# Autodesk Inventor assembly: rv_ledbrick_8ch
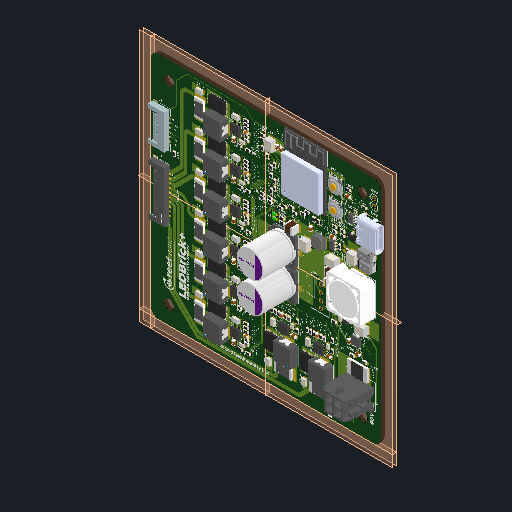
[picture p0: Inventor's stored thumbnail of the model, 512x512]
Saved by Autodesk Inventor 2026.1 (Build 301233020, 233B)
## iProperties
Created: 2025-09-11
Part Number: rv_ledbrick_8ch
Document SubType Name: Assembly
Designer: atrus
Author: atrus
## Documents named in this file (49)
- C:\Users\atrus\Dropbox\elec\Mechanical\LEDBrick\PCB\rv_ledbrick_8ch.iam
- C:\Users\atrus\Dropbox\elec\Mechanical\LEDBrick\PCB\rv_ledbrick_8ch_BOARD.ipt
- C:\Users\atrus\Dropbox\elec\Mechanical\LEDBrick\PCB\ConvertedComponents\LED_WS2812B2020_CMP-004-00042-1.ipt
- C:\Users\atrus\Dropbox\elec\Mechanical\LEDBrick\PCB\ConvertedComponents\RESC1608-IPC-ML_CMP-009-00193-3.ipt
- C:\Users\atrus\Dropbox\elec\Mechanical\LEDBrick\PCB\ConvertedComponents\SOT23-3_CMP-094-0000-1.ipt
- C:\Users\atrus\Dropbox\elec\Mechanical\LEDBrick\PCB\ConvertedComponents\RESC1608-IPC-LL_CMP-009-00205-1.ipt
- C:\Users\atrus\Dropbox\elec\Mechanical\LEDBrick\PCB\ConvertedComponents\RESC1608-IPC-NL_CMP-009-00180-2.ipt
- C:\Users\atrus\Dropbox\elec\Mechanical\LEDBrick\PCB\ConvertedComponents\RESC1608-IPC-ML_CMP-009-00191-4.ipt
- C:\Users\atrus\Dropbox\elec\Mechanical\LEDBrick\PCB\ConvertedComponents\RESC1608-IPC-NL_CMP-009-00191-4.ipt
- C:\Users\atrus\Dropbox\elec\Mechanical\LEDBrick\PCB\ConvertedComponents\FP-DGS0010A-IPC_C_CMP-015-00018-1.ipt
- C:\Users\atrus\Dropbox\elec\Mechanical\LEDBrick\PCB\ConvertedComponents\FP-RC0603-0_55-MFG_CMP-009-00246-1.ipt
- C:\Users\atrus\Dropbox\elec\Mechanical\LEDBrick\PCB\ConvertedComponents\RESC7146X09N_CMP-009-00241-2.ipt
- C:\Users\atrus\Dropbox\elec\Mechanical\LEDBrick\PCB\ConvertedComponents\FP-43045-0428-MFG_CMP-002-00096-1.ipt
- C:\Users\atrus\Dropbox\elec\Mechanical\LEDBrick\PCB\ConvertedComponents\FP-CL10-IPC_B_CMP-001-00084-7.ipt
- C:\Users\atrus\Dropbox\elec\Mechanical\LEDBrick\PCB\ConvertedComponents\LED-0603_CMP-130-0000-1.ipt
- C:\Users\atrus\Dropbox\elec\Mechanical\LEDBrick\PCB\ConvertedComponents\FP-504050-1091-MFG_CMP-002-00088-1.ipt
- C:\Users\atrus\Dropbox\elec\Mechanical\LEDBrick\PCB\ConvertedComponents\MOLEX_5040500691_CMP-253-000000-2.ipt
- C:\Users\atrus\Dropbox\elec\Mechanical\LEDBrick\PCB\ConvertedComponents\FP-OS-CON-SMT-F12-MFG_CMP-001-00120-1.ipt
- C:\Users\atrus\Dropbox\elec\Mechanical\LEDBrick\PCB\ConvertedComponents\SOT95P280X145-6N_CMP-019-00077-1.ipt
- C:\Users\atrus\Dropbox\elec\Mechanical\LEDBrick\PCB\ConvertedComponents\FP-DDC0006A-IPC_C_CMP-019-00081-1.ipt
- C:\Users\atrus\Dropbox\elec\Mechanical\LEDBrick\PCB\ConvertedComponents\XCVR_ESP32-S3-MINI-1-N8_CMP-247-000000-1.ipt
- C:\Users\atrus\Dropbox\elec\Mechanical\LEDBrick\PCB\ConvertedComponents\FP-PTS526SK15SMTR2LFS-MFG_CMP-011-00015-1.ipt
- C:\Users\atrus\Dropbox\elec\Mechanical\LEDBrick\PCB\ConvertedComponents\RESC1608X55X30NL20T20_CMP-009-00235-1.ipt
- C:\Users\atrus\Dropbox\elec\Mechanical\LEDBrick\PCB\ConvertedComponents\RESC1608-IPC-LL_CMP-009-00203-1.ipt
- C:\Users\atrus\Dropbox\elec\Mechanical\LEDBrick\PCB\ConvertedComponents\RESC1608-IPC-LL_CMP-009-00207-3.ipt
- C:\Users\atrus\Dropbox\elec\Mechanical\LEDBrick\PCB\ConvertedComponents\FP-AC0402-IPC_A_CMP-009-00234-1.ipt
- C:\Users\atrus\Dropbox\elec\Mechanical\LEDBrick\PCB\ConvertedComponents\SRR1260-680M-Footprint-1_CMP-006-00034-1.ipt
- C:\Users\atrus\Dropbox\elec\Mechanical\LEDBrick\PCB\ConvertedComponents\FP-SRN4018-MFG_CMP-006-00036-2.ipt
- C:\Users\atrus\Dropbox\elec\Mechanical\LEDBrick\PCB\ConvertedComponents\AMPHENOL_10155435-00011LF_CMP-243-000000-3.ipt
- C:\Users\atrus\Dropbox\elec\Mechanical\LEDBrick\PCB\ConvertedComponents\SMA_CMP-080-0002-2.ipt
- C:\Users\atrus\Dropbox\elec\Mechanical\LEDBrick\PCB\ConvertedComponents\FP-SOT23-6L-MFG_CMP-004-00040-1.ipt
- C:\Users\atrus\Dropbox\elec\Mechanical\LEDBrick\PCB\ConvertedComponents\CAPC3225X20N_CMP-001-00083-3.ipt
- C:\Users\atrus\Dropbox\elec\Mechanical\LEDBrick\PCB\ConvertedComponents\FP-1210-L_3_2_0_3-W_2_5_0-MFG_CMP-001-00125-1.ipt
- C:\Users\atrus\Dropbox\elec\Mechanical\LEDBrick\PCB\ConvertedComponents\CAPC1210(3225)230_M_CMP-001-00128-1.ipt
- C:\Users\atrus\Dropbox\elec\Mechanical\LEDBrick\PCB\ConvertedComponents\FP-GRM32E-0_2-0_3-MFG_CMP-001-00119-1.ipt
- C:\Users\atrus\Dropbox\elec\Mechanical\LEDBrick\PCB\ConvertedComponents\CAPC2013X94X50ML20T25_CMP-001-00130-1.ipt
- C:\Users\atrus\Dropbox\elec\Mechanical\LEDBrick\PCB\ConvertedComponents\FP-CL10-IPC_B_CMP-001-00085-7.ipt
- C:\Users\atrus\Dropbox\elec\Mechanical\LEDBrick\PCB\ConvertedComponents\RESC1608-IPC-NL_CMP-009-00208-2.ipt
- C:\Users\atrus\Dropbox\elec\Mechanical\LEDBrick\PCB\ConvertedComponents\SON50P300X100_HS-13N_CMP-019-00085-2.ipt
- C:\Users\atrus\Dropbox\elec\Mechanical\LEDBrick\PCB\ConvertedComponents\RESC1608-IPC-NL_CMP-009-00203-1.ipt
- C:\Users\atrus\Dropbox\elec\Mechanical\LEDBrick\PCB\ConvertedComponents\RESC1608X55X30ML15T15_CMP-009-00245-1.ipt
- C:\Users\atrus\Dropbox\elec\Mechanical\LEDBrick\PCB\ConvertedComponents\FP-CRCW0603-e3-IPC_B_CMP-009-00244-2.ipt
- C:\Users\atrus\Dropbox\elec\Mechanical\LEDBrick\PCB\ConvertedComponents\RESC1608-IPC-NL_CMP-009-00187-4.ipt
- C:\Users\atrus\Dropbox\elec\Mechanical\LEDBrick\PCB\ConvertedComponents\RESC1608-IPC-NL_CMP-009-00193-3.ipt
- C:\Users\atrus\Dropbox\elec\Mechanical\LEDBrick\PCB\ConvertedComponents\FP-CRA2512-MFG_CMP-009-00243-1.ipt
- C:\Users\atrus\Dropbox\elec\Mechanical\LEDBrick\PCB\ConvertedComponents\FP-IHLP-2525CZ-FP_2_413x3-MFG_CMP-006-00037-1.ipt
- C:\Users\atrus\Dropbox\elec\Mechanical\LEDBrick\PCB\ConvertedComponents\DFN355P580X82-3N_CMP-004-00041-2.ipt
- C:\Users\atrus\Dropbox\elec\Mechanical\LEDBrick\PCB\ConvertedComponents\FP-0603-L_1_6_0_15-W_0_81-IPC_B_CMP-001-00131-2.ipt
- C:\Users\atrus\Dropbox\elec\Mechanical\LEDBrick\PCB\ConvertedComponents\CAPC2013X94X50NL20T25_CMP-001-00130-1.ipt
## Components (210 placed, 210 different names)
1. rv_ledbrick_8ch_BOARD:1 — Symmetry:1, Symmetry:2
2. LED_WS2812B2020_CMP-004-00042-1:1{D200}
3. RESC1608-IPC-ML_CMP-009-00193-3:1{R230}
4. RESC1608-IPC-ML_CMP-009-00193-3:2{R205}
5. RESC1608-IPC-ML_CMP-009-00193-3:3{R206}
6. SOT23-3_CMP-094-0000-1:1{Q201}
7. SOT23-3_CMP-094-0000-1:2{Q200}
8. RESC1608-IPC-LL_CMP-009-00205-1:1{R10}
9. RESC1608-IPC-NL_CMP-009-00180-2:1{R229}
10. RESC1608-IPC-NL_CMP-009-00180-2:2{R228}
11. RESC1608-IPC-NL_CMP-009-00180-2:3{R224}
12. RESC1608-IPC-NL_CMP-009-00180-2:4{R9_H}
13. RESC1608-IPC-NL_CMP-009-00180-2:5{R9_G}
14. RESC1608-IPC-NL_CMP-009-00180-2:6{R9_F}
15. RESC1608-IPC-NL_CMP-009-00180-2:7{R9_E}
16. RESC1608-IPC-NL_CMP-009-00180-2:8{R9_D}
17. RESC1608-IPC-NL_CMP-009-00180-2:9{R9_C}
18. RESC1608-IPC-NL_CMP-009-00180-2:10{R9_B}
19. RESC1608-IPC-NL_CMP-009-00180-2:11{R9_A}
20. RESC1608-IPC-NL_CMP-009-00180-2:12{R8_H}
21. RESC1608-IPC-NL_CMP-009-00180-2:13{R8_G}
22. RESC1608-IPC-NL_CMP-009-00180-2:14{R8_F}
23. RESC1608-IPC-NL_CMP-009-00180-2:15{R8_E}
24. RESC1608-IPC-NL_CMP-009-00180-2:16{R8_D}
25. RESC1608-IPC-NL_CMP-009-00180-2:17{R8_C}
26. RESC1608-IPC-NL_CMP-009-00180-2:18{R8_B}
27. RESC1608-IPC-NL_CMP-009-00180-2:19{R8_A}
28. RESC1608-IPC-ML_CMP-009-00191-4:1{R227}
29. RESC1608-IPC-ML_CMP-009-00191-4:2{R226}
30. RESC1608-IPC-ML_CMP-009-00191-4:3{R223}
31. RESC1608-IPC-ML_CMP-009-00191-4:4{R222}
32. RESC1608-IPC-ML_CMP-009-00191-4:5{R221}
33. RESC1608-IPC-ML_CMP-009-00191-4:6{R204}
34. RESC1608-IPC-ML_CMP-009-00191-4:7{R202}
35. RESC1608-IPC-ML_CMP-009-00191-4:8{R201}
36. RESC1608-IPC-NL_CMP-009-00191-4:1{R225}
37. RESC1608-IPC-NL_CMP-009-00191-4:2{R220}
38. RESC1608-IPC-NL_CMP-009-00191-4:3{R219}
39. RESC1608-IPC-NL_CMP-009-00191-4:4{R218}
40. RESC1608-IPC-NL_CMP-009-00191-4:5{R217}
41. RESC1608-IPC-NL_CMP-009-00191-4:6{R216}
42. RESC1608-IPC-NL_CMP-009-00191-4:7{R215}
43. RESC1608-IPC-NL_CMP-009-00191-4:8{R214}
44. RESC1608-IPC-NL_CMP-009-00191-4:9{R213}
45. RESC1608-IPC-NL_CMP-009-00191-4:10{R212}
46. RESC1608-IPC-NL_CMP-009-00191-4:11{R211}
47. RESC1608-IPC-NL_CMP-009-00191-4:12{R210}
48. RESC1608-IPC-NL_CMP-009-00191-4:13{R209}
49. RESC1608-IPC-NL_CMP-009-00191-4:14{R208}
50. RESC1608-IPC-NL_CMP-009-00191-4:15{R207}
51. RESC1608-IPC-NL_CMP-009-00191-4:16{R203}
52. RESC1608-IPC-NL_CMP-009-00191-4:17{R200}
53. FP-DGS0010A-IPC_C_CMP-015-00018-1:1{U500}
54. FP-RC0603-0_55-MFG_CMP-009-00246-1:1{R502}
55. FP-RC0603-0_55-MFG_CMP-009-00246-1:2{R500}
56. RESC7146X09N_CMP-009-00241-2:1{R501}
57. FP-43045-0428-MFG_CMP-002-00096-1:1{J500}
58. FP-CL10-IPC_B_CMP-001-00084-7:1{C501}
59. FP-CL10-IPC_B_CMP-001-00084-7:2{C500}
60. FP-CL10-IPC_B_CMP-001-00084-7:3{C404}
61. FP-CL10-IPC_B_CMP-001-00084-7:4{C401}
62. FP-CL10-IPC_B_CMP-001-00084-7:5{C201}
63. FP-CL10-IPC_B_CMP-001-00084-7:6{C200}
64. LED-0603_CMP-130-0000-1:1{LED201}
65. LED-0603_CMP-130-0000-1:2{LED200}
66. FP-504050-1091-MFG_CMP-002-00088-1:1{J4}
67. FP-504050-1091-MFG_CMP-002-00088-1:2{J1}
68. MOLEX_5040500691_CMP-253-000000-2:1{J3}
69. FP-OS-CON-SMT-F12-MFG_CMP-001-00120-1:1{C6}
70. FP-OS-CON-SMT-F12-MFG_CMP-001-00120-1:2{C5}
71. SOT95P280X145-6N_CMP-019-00077-1:1{U400}
72. FP-DDC0006A-IPC_C_CMP-019-00081-1:1{U401}
73. XCVR_ESP32-S3-MINI-1-N8_CMP-247-000000-1:1{U200}
74. FP-PTS526SK15SMTR2LFS-MFG_CMP-011-00015-1:1{RST200}
75. FP-PTS526SK15SMTR2LFS-MFG_CMP-011-00015-1:2{BOOT200}
76. RESC1608X55X30NL20T20_CMP-009-00235-1:1{R402}
77. RESC1608-IPC-LL_CMP-009-00203-1:1{R400}
78. RESC1608-IPC-LL_CMP-009-00203-1:2{R401}
79. RESC1608-IPC-LL_CMP-009-00207-3:1{R403}
80. FP-AC0402-IPC_A_CMP-009-00234-1:1{R301}
81. FP-AC0402-IPC_A_CMP-009-00234-1:2{R300}
82. SRR1260-680M-Footprint-1_CMP-006-00034-1:1{L400}
83. FP-SRN4018-MFG_CMP-006-00036-2:1{L401}
84. AMPHENOL_10155435-00011LF_CMP-243-000000-3:1{J300}
85. SMA_CMP-080-0002-2:1{D401}
86. SMA_CMP-080-0002-2:2{D400}
87. FP-SOT23-6L-MFG_CMP-004-00040-1:1{D300}
88. CAPC3225X20N_CMP-001-00083-3:1{C410}
89. CAPC3225X20N_CMP-001-00083-3:2{C402}
90. CAPC3225X20N_CMP-001-00083-3:3{C405}
91. CAPC3225X20N_CMP-001-00083-3:4{C202}
92. FP-1210-L_3_2_0_3-W_2_5_0-MFG_CMP-001-00125-1:1{C409}
93. FP-1210-L_3_2_0_3-W_2_5_0-MFG_CMP-001-00125-1:2{C403}
94. CAPC1210(3225)230_M_CMP-001-00128-1:1{C406}
95. FP-GRM32E-0_2-0_3-MFG_CMP-001-00119-1:1{C407}
96. CAPC2013X94X50ML20T25_CMP-001-00130-1:1{C400}
97. FP-CL10-IPC_B_CMP-001-00085-7:1{C206}
98. FP-CL10-IPC_B_CMP-001-00085-7:2{C203}
99. FP-CL10-IPC_B_CMP-001-00085-7:3{C2_H}
100. FP-CL10-IPC_B_CMP-001-00085-7:4{C2_G}
101. FP-CL10-IPC_B_CMP-001-00085-7:5{C2_F}
102. FP-CL10-IPC_B_CMP-001-00085-7:6{C2_E}
103. FP-CL10-IPC_B_CMP-001-00085-7:7{C2_D}
104. FP-CL10-IPC_B_CMP-001-00085-7:8{C2_C}
105. FP-CL10-IPC_B_CMP-001-00085-7:9{C2_B}
106. FP-CL10-IPC_B_CMP-001-00085-7:10{C2_A}
107. RESC1608-IPC-NL_CMP-009-00208-2:1{R4_F}
108. RESC1608-IPC-NL_CMP-009-00208-2:2{R4_H}
109. RESC1608-IPC-NL_CMP-009-00208-2:3{R4_G}
110. RESC1608-IPC-NL_CMP-009-00208-2:4{R4_E}
111. RESC1608-IPC-NL_CMP-009-00208-2:5{R4_D}
112. RESC1608-IPC-NL_CMP-009-00208-2:6{R4_C}
113. RESC1608-IPC-NL_CMP-009-00208-2:7{R4_B}
114. RESC1608-IPC-NL_CMP-009-00208-2:8{R4_A}
115. SON50P300X100_HS-13N_CMP-019-00085-2:1{U1_H}
116. SON50P300X100_HS-13N_CMP-019-00085-2:2{U1_G}
117. SON50P300X100_HS-13N_CMP-019-00085-2:3{U1_F}
118. SON50P300X100_HS-13N_CMP-019-00085-2:4{U1_E}
119. SON50P300X100_HS-13N_CMP-019-00085-2:5{U1_D}
120. SON50P300X100_HS-13N_CMP-019-00085-2:6{U1_C}
121. SON50P300X100_HS-13N_CMP-019-00085-2:7{U1_B}
122. SON50P300X100_HS-13N_CMP-019-00085-2:8{U1_A}
123. RESC1608-IPC-NL_CMP-009-00203-1:1{R7_H}
124. RESC1608-IPC-NL_CMP-009-00203-1:2{R7_G}
125. RESC1608-IPC-NL_CMP-009-00203-1:3{R7_F}
126. RESC1608-IPC-NL_CMP-009-00203-1:4{R7_E}
127. RESC1608-IPC-NL_CMP-009-00203-1:5{R7_D}
128. RESC1608-IPC-NL_CMP-009-00203-1:6{R7_C}
129. RESC1608-IPC-NL_CMP-009-00203-1:7{R7_B}
130. RESC1608-IPC-NL_CMP-009-00203-1:8{R7_A}
131. RESC1608X55X30ML15T15_CMP-009-00245-1:1{R6_H}
132. RESC1608X55X30ML15T15_CMP-009-00245-1:2{R6_G}
133. RESC1608X55X30ML15T15_CMP-009-00245-1:3{R6_F}
134. RESC1608X55X30ML15T15_CMP-009-00245-1:4{R6_E}
135. RESC1608X55X30ML15T15_CMP-009-00245-1:5{R6_D}
136. RESC1608X55X30ML15T15_CMP-009-00245-1:6{R6_C}
137. RESC1608X55X30ML15T15_CMP-009-00245-1:7{R6_B}
138. RESC1608X55X30ML15T15_CMP-009-00245-1:8{R6_A}
139. FP-CRCW0603-e3-IPC_B_CMP-009-00244-2:1{R5_H}
140. FP-CRCW0603-e3-IPC_B_CMP-009-00244-2:2{R5_G}
141. FP-CRCW0603-e3-IPC_B_CMP-009-00244-2:3{R5_F}
142. FP-CRCW0603-e3-IPC_B_CMP-009-00244-2:4{R5_E}
143. FP-CRCW0603-e3-IPC_B_CMP-009-00244-2:5{R5_D}
144. FP-CRCW0603-e3-IPC_B_CMP-009-00244-2:6{R5_C}
145. FP-CRCW0603-e3-IPC_B_CMP-009-00244-2:7{R5_B}
146. FP-CRCW0603-e3-IPC_B_CMP-009-00244-2:8{R5_A}
147. RESC1608-IPC-NL_CMP-009-00187-4:1{R3_H}
148. RESC1608-IPC-NL_CMP-009-00187-4:2{R3_G}
149. RESC1608-IPC-NL_CMP-009-00187-4:3{R3_F}
150. RESC1608-IPC-NL_CMP-009-00187-4:4{R3_E}
151. RESC1608-IPC-NL_CMP-009-00187-4:5{R3_D}
152. RESC1608-IPC-NL_CMP-009-00187-4:6{R3_C}
153. RESC1608-IPC-NL_CMP-009-00187-4:7{R3_B}
154. RESC1608-IPC-NL_CMP-009-00187-4:8{R3_A}
155. RESC1608-IPC-NL_CMP-009-00193-3:1{R2_H}
156. RESC1608-IPC-NL_CMP-009-00193-3:2{R2_G}
157. RESC1608-IPC-NL_CMP-009-00193-3:3{R2_F}
158. RESC1608-IPC-NL_CMP-009-00193-3:4{R2_E}
159. RESC1608-IPC-NL_CMP-009-00193-3:5{R2_D}
160. RESC1608-IPC-NL_CMP-009-00193-3:6{R2_C}
161. RESC1608-IPC-NL_CMP-009-00193-3:7{R2_B}
162. RESC1608-IPC-NL_CMP-009-00193-3:8{R2_A}
163. FP-CRA2512-MFG_CMP-009-00243-1:1{R1_H}
164. FP-CRA2512-MFG_CMP-009-00243-1:2{R1_G}
165. FP-CRA2512-MFG_CMP-009-00243-1:3{R1_F}
166. FP-CRA2512-MFG_CMP-009-00243-1:4{R1_E}
167. FP-CRA2512-MFG_CMP-009-00243-1:5{R1_D}
168. FP-CRA2512-MFG_CMP-009-00243-1:6{R1_C}
169. FP-CRA2512-MFG_CMP-009-00243-1:7{R1_B}
170. FP-CRA2512-MFG_CMP-009-00243-1:8{R1_A}
171. FP-IHLP-2525CZ-FP_2_413x3-MFG_CMP-006-00037-1:1{L1_H}
172. FP-IHLP-2525CZ-FP_2_413x3-MFG_CMP-006-00037-1:2{L1_G}
173. FP-IHLP-2525CZ-FP_2_413x3-MFG_CMP-006-00037-1:3{L1_F}
174. FP-IHLP-2525CZ-FP_2_413x3-MFG_CMP-006-00037-1:4{L1_E}
175. FP-IHLP-2525CZ-FP_2_413x3-MFG_CMP-006-00037-1:5{L1_D}
176. FP-IHLP-2525CZ-FP_2_413x3-MFG_CMP-006-00037-1:6{L1_C}
177. FP-IHLP-2525CZ-FP_2_413x3-MFG_CMP-006-00037-1:7{L1_B}
178. FP-IHLP-2525CZ-FP_2_413x3-MFG_CMP-006-00037-1:8{L1_A}
179. DFN355P580X82-3N_CMP-004-00041-2:1{D1_H}
180. DFN355P580X82-3N_CMP-004-00041-2:2{D1_G}
181. DFN355P580X82-3N_CMP-004-00041-2:3{D1_F}
182. DFN355P580X82-3N_CMP-004-00041-2:4{D1_E}
183. DFN355P580X82-3N_CMP-004-00041-2:5{D1_D}
184. DFN355P580X82-3N_CMP-004-00041-2:6{D1_C}
185. DFN355P580X82-3N_CMP-004-00041-2:7{D1_B}
186. DFN355P580X82-3N_CMP-004-00041-2:8{D1_A}
187. FP-0603-L_1_6_0_15-W_0_81-IPC_B_CMP-001-00131-2:1{C4_H}
188. FP-0603-L_1_6_0_15-W_0_81-IPC_B_CMP-001-00131-2:2{C4_G}
189. FP-0603-L_1_6_0_15-W_0_81-IPC_B_CMP-001-00131-2:3{C4_F}
190. FP-0603-L_1_6_0_15-W_0_81-IPC_B_CMP-001-00131-2:4{C4_E}
191. FP-0603-L_1_6_0_15-W_0_81-IPC_B_CMP-001-00131-2:5{C4_D}
192. FP-0603-L_1_6_0_15-W_0_81-IPC_B_CMP-001-00131-2:6{C4_C}
193. FP-0603-L_1_6_0_15-W_0_81-IPC_B_CMP-001-00131-2:7{C4_B}
194. FP-0603-L_1_6_0_15-W_0_81-IPC_B_CMP-001-00131-2:8{C4_A}
195. CAPC2013X94X50NL20T25_CMP-001-00130-1:1{C3_H}
196. CAPC2013X94X50NL20T25_CMP-001-00130-1:2{C3_G}
197. CAPC2013X94X50NL20T25_CMP-001-00130-1:3{C3_F}
198. CAPC2013X94X50NL20T25_CMP-001-00130-1:4{C3_E}
199. CAPC2013X94X50NL20T25_CMP-001-00130-1:5{C3_D}
200. CAPC2013X94X50NL20T25_CMP-001-00130-1:6{C3_C}
201. CAPC2013X94X50NL20T25_CMP-001-00130-1:7{C3_B}
202. CAPC2013X94X50NL20T25_CMP-001-00130-1:8{C3_A}
203. CAPC2013X94X50NL20T25_CMP-001-00130-1:9{C1_H}
204. CAPC2013X94X50NL20T25_CMP-001-00130-1:10{C1_G}
205. CAPC2013X94X50NL20T25_CMP-001-00130-1:11{C1_F}
206. CAPC2013X94X50NL20T25_CMP-001-00130-1:12{C1_E}
207. CAPC2013X94X50NL20T25_CMP-001-00130-1:13{C1_D}
208. CAPC2013X94X50NL20T25_CMP-001-00130-1:14{C1_C}
209. CAPC2013X94X50NL20T25_CMP-001-00130-1:15{C1_B}
210. CAPC2013X94X50NL20T25_CMP-001-00130-1:16{C1_A}
## Relationships (2: Symmetry 2)
- Symmetry:1: rv_ledbrick_8ch_BOARD:1
- Symmetry:2: rv_ledbrick_8ch_BOARD:1
